# Autodesk Inventor assembly: Re-entrant Flange
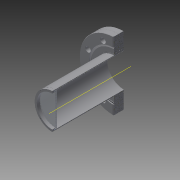
[picture p0: Inventor's stored thumbnail of the model, 180x180]
Saved by Autodesk Inventor 2015 (Build 190159000, 159)
## iProperties
Created: 2014-07-08
Part Number: Re-entrant Flange
Document SubType Name: Assembly
Designer: I Rabey
Author: I Rabey
## Documents named in this file (7)
- C:\ColdMatter\CADFiles\EDM Machine\Microwave Detection Region\Re-entrant Flange\Re-entrant Flange.iam
- C:\ColdMatter\CADFiles\EDM Machine\Microwave Detection Region\Re-entrant Flange\Vacuum Cylinder.ipt
- C:\ColdMatter\CADFiles\EDM Machine\Microwave Detection Region\Re-entrant Flange\DN63CF Counter Bored.ipt
- C:\ColdMatter\CADFiles\EDM Machine\Microwave Detection Region\Re-entrant Flange\Window.ipt
- C:\ColdMatter\CADFiles\EDM Machine\Microwave Detection Region\Re-entrant Flange\Cap.ipt
- C:\ColdMatter\CADFiles\EDM Machine\Microwave Detection Region\Re-entrant Flange\ORing537ID.ipt
- C:\ColdMatter\CADFiles\EDM Machine\Microwave Detection Region\Re-entrant Flange\Lens Ring.ipt
## Components (6 placed, 6 different names)
1. DN63CF Counter Bored:1 — Mate:1, Mate:2, Mate:3, Mate:4
2. Vacuum Cylinder:1 — Mate:3, Mate:4, Mate:5, Mate:6, Mate:9
3. Window:1 — Mate:5, Mate:6, Mate:10, Mate:12
4. Cap:1 — Mate:7, Mate:8, Mate:9, Angle:1, Mate:11
5. ORing537ID:1 — Mate:7, Mate:8, Mate:10
6. Lens Ring:1 — Mate:11, Mate:12
## Relationships (13: Mate 12, Angle 1)
- Mate:1: DN63CF Counter Bored:1
- Mate:2: DN63CF Counter Bored:1
- Mate:3: DN63CF Counter Bored:1 ↔ Vacuum Cylinder:1
- Mate:4: DN63CF Counter Bored:1 ↔ Vacuum Cylinder:1
- Mate:5: Vacuum Cylinder:1 ↔ Window:1
- Mate:6: Vacuum Cylinder:1 ↔ Window:1
- Mate:7: Cap:1 ↔ ORing537ID:1
- Mate:8: Cap:1 ↔ ORing537ID:1
- Mate:9: Vacuum Cylinder:1 ↔ Cap:1
- Mate:10: Window:1 ↔ ORing537ID:1
- Angle:1 (45 deg): Cap:1
- Mate:11: Cap:1 ↔ Lens Ring:1
- Mate:12: Window:1 ↔ Lens Ring:1
